# Autodesk Inventor assembly: Lever Arm
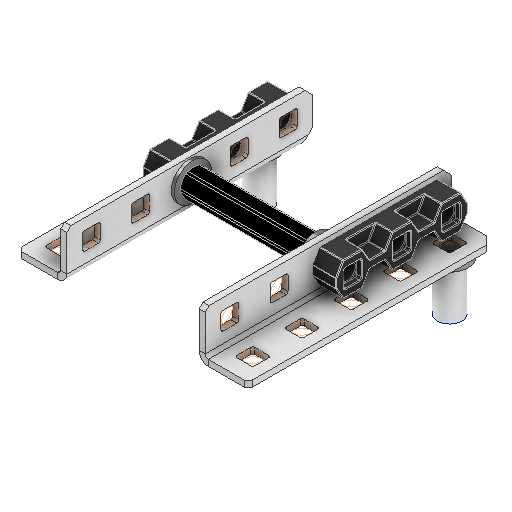
[picture p0: Inventor's stored thumbnail of the model, 512x512]
Saved by Autodesk Inventor 2025 (Build 290162000, 162)
## iProperties
Created: 2025-02-15
Part Number: Lever Arm
Document SubType Name: Assembly
Designer: Averey Ku
Author: Averey Ku
## Documents named in this file (8)
- D:\VEX\High Stakes\CAD\V5\Clamp\Lever Arm.iam
- D:\VEX\High Stakes\CAD\ROBOPROS-CAD-Inventor\Structure\Angle\Aluminum 1x1\Alu Angle 1x1x5.ipt
- D:\VEX\High Stakes\CAD\ROBOPROS-CAD-Inventor\Motion\Shaft LS\Bearing Flat Low Profile.ipt
- D:\VEX\High Stakes\CAD\ROBOPROS-CAD-Inventor\Structure\Standoff\Standoff 1.25.ipt
- D:\VEX\High Stakes\CAD\ROBOPROS-CAD-Inventor\Motion\Spacers\Washer Steel\SWasher .375 OD x .031250.ipt
- D:\VEX\High Stakes\CAD\ROBOPROS-CAD-Inventor\Motion\Spacers\Washer Steel.ipt
- D:\VEX\High Stakes\CAD\ROBOPROS-CAD-Inventor\Motion\Spacers\Washer Steel\SWasher .375 OD x .062500.ipt
- D:\VEX\High Stakes\CAD\ROBOPROS-CAD-Inventor\Structure\Standoff Rounded\Standoff Rounded .500.ipt
## Components (11 placed, 6 different names)
1. Alu Angle 1x1x5:1 — Mate:1, Flush:1, Mate:3, Insert:1, Mate:4, Insert:7
2. Alu Angle 1x1x5:2 — Flush:2, Mate:2, Flush:3, Insert:2, Mate:5, Insert:5, Insert:9
3. Bearing Flat Low Profile:1 — Insert:2, Mate:5
4. Bearing Flat Low Profile:2 — Insert:1, Mate:4
5. Standoff 1.25:1 — Insert:3, Insert:4
6. SWasher .375 OD x .031250:1 — Insert:4, Insert:5
7. SWasher .375 OD x .062500:2 — Insert:3
8. SWasher .375 OD x .062500:3 — Insert:6, Insert:7
9. Standoff Rounded .500:1 — Insert:6
10. SWasher .375 OD x .062500:4 — Insert:9
11. Standoff Rounded .500:2
## Relationships (17: Insert 9, Mate 5, Flush 3)
- Mate:1: Alu Angle 1x1x5:1
- Flush:1 (-31.75 mm): Alu Angle 1x1x5:1
- Flush:2 (-31.75 mm): Alu Angle 1x1x5:2
- Mate:2: Alu Angle 1x1x5:2
- Mate:3 (17.0656 mm): Alu Angle 1x1x5:1
- Flush:3 (17.0656 mm): Alu Angle 1x1x5:2
- Insert:1: Alu Angle 1x1x5:1 ↔ Bearing Flat Low Profile:2
- Mate:4: Alu Angle 1x1x5:1 ↔ Bearing Flat Low Profile:2
- Insert:2: Alu Angle 1x1x5:2 ↔ Bearing Flat Low Profile:1
- Mate:5: Alu Angle 1x1x5:2 ↔ Bearing Flat Low Profile:1
- Insert:3: Standoff 1.25:1 ↔ SWasher .375 OD x .062500:2
- Insert:4: Standoff 1.25:1 ↔ SWasher .375 OD x .031250:1
- Insert:5: Alu Angle 1x1x5:2 ↔ SWasher .375 OD x .031250:1
- Insert:6: SWasher .375 OD x .062500:3 ↔ Standoff Rounded .500:1
- Insert:7: Alu Angle 1x1x5:1 ↔ SWasher .375 OD x .062500:3
- [Insert]: SWasher .375 OD x .062500:4 ↔ Standoff Rounded .500:2
- Insert:9: Alu Angle 1x1x5:2 ↔ SWasher .375 OD x .062500:4
## Named parameters: d15_d13 = 0 mm
